# Autodesk Inventor assembly: 36-tooth Differential Assembly
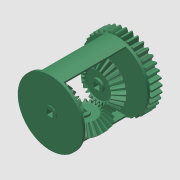
[picture p0: Inventor's stored thumbnail of the model, 180x180]
Saved by Autodesk Inventor 2020 (Build 240168000, 168)
## iProperties
Document SubType Name: Assembly
Designer: Jordan Kiesel
Description: Create more efficient "car style" drivetrains.
Vendor: VEX Robotics, Inc.
Catalog Web Link: vexrobotics.com/276-2184.html
Created: 2019-05-18
Category: Motion
Company: Super Sonic Sparks, Team 24
Translation Standard: STEP AP203
FileName: 36-tooth Differential Assembly.iam
PreProcessor: SolidWorks 2006052
PostProcessor: Build: 239, Release: 2011 RTM - Date: Wed 02/17/2010
Sent Units: inch
Uncertainty: 1e-05
Author: Jordan Kiesel
Title: 36-tooth Differential Assembly
Comments: This can be utilized to create more efficient "car style" drivetrains.
## Documents named in this file (3)
- D:\Valut\ncrCadLib\高级力学套件\36-Tooth Differential Assembly.iam
- D:\Valut\ncrCadLib\高级力学套件\24-Tooth Bevel Gear.ipt
- D:\Valut\ncrCadLib\高级力学套件\Reference Parts\36-Tooth Differential Assembly\36-Tooth Differential Housing.ipt
## Components (4 placed, 2 different names)
1. 24-Tooth Bevel Gear:1 — Insert:1, Rotation:1
2. 36-Tooth Differential Housing:1 — Insert:1, Insert:2, Insert:3
3. 24-Tooth Bevel Gear:2 — Insert:2, Rotation:2
4. 24-Tooth Bevel Gear:3 — Insert:3, Rotation:1, Rotation:2
## Relationships (5: Insert 3, RelateRotation 2)
- Insert:1: 24-Tooth Bevel Gear:1 ↔ 36-Tooth Differential Housing:1
- Insert:2: 36-Tooth Differential Housing:1 ↔ 24-Tooth Bevel Gear:2
- Insert:3: 36-Tooth Differential Housing:1 ↔ 24-Tooth Bevel Gear:3
- Rotation:1 [RelateRotation] (1 ul): 24-Tooth Bevel Gear:1 ↔ 24-Tooth Bevel Gear:3
- Rotation:2 [RelateRotation] (1 ul): 24-Tooth Bevel Gear:2 ↔ 24-Tooth Bevel Gear:3
